# Autodesk Inventor assembly: hoops_sml_med_lrg
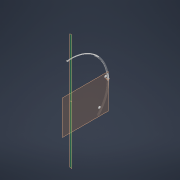
[picture p0: Inventor's stored thumbnail of the model, 180x180]
Saved by Autodesk Inventor 2021 (Build 250183000, 183)
## iProperties
Created: 2021-05-05
Part Number: hoops_sml_med_lrg
Document SubType Name: Assembly
## Documents named in this file (11)
- C:\Users\Watchdog\OneDrive - Flinders\Advn Mech Design Shared\6_Development\2_Design\inventor\Brandon_Hoop_specs\hoops_sml_med_lrg.iam
- C:\Users\Watchdog\OneDrive - Flinders\Advn Mech Design Shared\6_Development\2_Design\inventor\Brandon_Hoop_specs\large_hoop.ipt
- C:\Users\Watchdog\OneDrive - Flinders\Advn Mech Design Shared\6_Development\2_Design\inventor\Brandon_Hoop_specs\medium_hoop.ipt
- C:\Users\Watchdog\OneDrive - Flinders\Advn Mech Design Shared\6_Development\2_Design\inventor\rack_pinion\pinion.ipt
- C:\Users\Watchdog\OneDrive - Flinders\Advn Mech Design Shared\6_Development\2_Design\inventor\Brandon_Hoop_specs\small_hoop.ipt
- C:\Users\Watchdog\OneDrive - Flinders\Advn Mech Design Shared\6_Development\2_Design\inventor\rack_pinion\tooth.ipt
- C:\Users\Watchdog\OneDrive - Flinders\Advn Mech Design Shared\6_Development\2_Design\inventor\rack_pinion\pulley_guide.ipt
- C:\Users\Watchdog\OneDrive - Flinders\Advn Mech Design Shared\6_Development\2_Design\inventor\rack_pinion\large_bearings.ipt
- C:\Users\Watchdog\OneDrive - Flinders\Advn Mech Design Shared\6_Development\2_Design\inventor\rack_pinion\medium_bearings.ipt
- C:\Users\Watchdog\OneDrive - Flinders\Advn Mech Design Shared\6_Development\2_Design\inventor\rack_pinion\medium_pulley.ipt
- C:\Users\Watchdog\OneDrive - Flinders\Advn Mech Design Shared\6_Development\2_Design\inventor\params.xlsx
## Components (69 placed, 9 different names)
1. large_hoop:1 — Mate:1, Flush:1, Flush:12, Angle:1
2. medium_hoop:1 — Mate:2, Flush:2, Mate:4, Flush:8, Flush:9, Mate:6, Mate:7, Mate:12
3. pinion:1 — Flush:6
4. small_hoop:1 — Mate:3, Flush:7, Mate:8, Mate:9
5. large_bearings:1 — Mate:6, Flush:12
6. medium_bearings:1 — Flush:13, Mate:7
7. pinion:2
8. pulley_guide:1 — Mate:8, Mate:9, Mate:10
9. medium_pulley:1 — Mate:11, Mate:12
10. tooth:1 — Mate:4, Flush:8, Flush:9
11. tooth:2
12. tooth:3
13. tooth:4
14. tooth:5
15. tooth:6
16. tooth:7
17. tooth:8
18. tooth:9
19. tooth:10
20. tooth:11
21. tooth:12
22. tooth:13
23. tooth:14
24. tooth:15
25. tooth:16
26. tooth:17
27. tooth:18
28. tooth:19
29. tooth:20
30. tooth:21
31. tooth:22
32. tooth:23
33. tooth:24
34. tooth:25
35. tooth:26
36. tooth:27
37. tooth:28
38. tooth:29
39. tooth:30
40. tooth:31
41. tooth:32
42. tooth:33
43. tooth:34
44. tooth:35
45. tooth:36
46. tooth:37
47. tooth:38
48. tooth:39
49. tooth:40
50. tooth:41
51. tooth:42
52. tooth:43
53. tooth:44
54. tooth:45
55. tooth:46
56. tooth:47
57. tooth:48
58. tooth:49
59. tooth:50
60. tooth:51
61. tooth:52
62. tooth:53
63. tooth:54
64. tooth:55
65. tooth:56
66. tooth:57
67. tooth:58
68. tooth:59
69. tooth:60
## Component patterns: (60 elements, first: tooth:1)
## Relationships (21: Mate 11, Flush 9, Angle 1)
- Mate:1: large_hoop:1
- Mate:2: medium_hoop:1
- Flush:1: large_hoop:1
- Flush:2: medium_hoop:1
- Flush:6: pinion:1
- Mate:3: small_hoop:1
- Flush:7: small_hoop:1
- Mate:4: medium_hoop:1 ↔ tooth:1
- Flush:8: medium_hoop:1 ↔ tooth:1
- Flush:9: medium_hoop:1 ↔ tooth:1
- Mate:6: medium_hoop:1 ↔ large_bearings:1
- Flush:12: large_hoop:1 ↔ large_bearings:1
- Flush:13: medium_bearings:1
- Mate:7: medium_hoop:1 ↔ medium_bearings:1
- Mate:8 (-10 mm): small_hoop:1 ↔ pulley_guide:1
- Mate:9: small_hoop:1 ↔ pulley_guide:1
- Mate:10: pulley_guide:1
- Mate:11: medium_pulley:1
- Mate:12: medium_hoop:1 ↔ medium_pulley:1
- Flush:14
- Angle:1 (180 deg): large_hoop:1
## Named parameters: testLength = 1700 mm, testWidth = 1500 mm, testHeight = 1000 mm, rack_tooth_thickness = 5 mm, rack_tooth_face_widh = 10 mm, rack_tooth_addendum = 5 mm, rack_tooth_dedendum = 5 mm, hoop_radius_large = 3300 mm, hoop_width_large = 80 mm, hoop_thickness_large = 10 mm, hoop_width_medium = 60 mm, hoop_thickness_medium = 10 mm, hoop_width_small = 40 mm, hoop_thickness_small = 10 mm, hoop_height_large = 450 mm, hoop_height_medium = 450 mm, hoop_height_small = 600 mm, hoop_length_large = 200 mm, hoop_length_medium = 700 mm, hoop_length_small = 700 mm, cover_width_main = 1600 mm, cover_height_main = 900 mm, cover_length_main = 2200 mm, cover_shell_thickness = 10 mm, cover_base_thickness = 10 mm, cover_mountHole_diameter = 10 mm, cover_mountHole_xSpacing = 900 mm, cover_mountHole_ySpacing = 550 mm, cover_side_thickness = 20 mm, cover_side_openSize = 1400 mm, hoop_bearing_length = 5 deg, hoop_cable_diam = 5 mm, hoop_cable_pulley_diam = 22 mm, secure_arm_length = 400 mm, secure_arm_radii = 9 mm, secure_arm_hold_length = 35 mm, secure_arm_hold_thickness = 10 mm, secure_arm_thickness = 20 mm, secure_arm_angle = 20 deg, support_frame_squareBarThickness = 5 mm, support_frame_squareBarDimension = 50 mm, support_frame_squareBarFillet = 2 mm, support_baseClamp_platformThickness = 15 mm, support_baseClamp_sleeve_hole2Height = 100 mm, support_baseClamp_platformWidthBuffer = 0 mm, support_baseClamp_sleeveThickness = 20 mm, support_baseClamp_platformLengthBuffer = 35 mm, support_baseClamp_sleeve_hole1Height = 50 mm, support_frame_length = 500 mm, support_frame_endHoleBuffer = 25 mm, support_frame_clampHoleSpacing = 100 mm, support_frame_clampHoleDiameter = 10 mm, support_baseClamp_thickness = 8 mm, support_baseClamp_sleeveSweepTerminationAngle = 55 deg, support_baseClamp_sleeveHoleDiameter = 12 mm, support_baseClamp_lengthBuffer = 40 mm, hoop_offset_x = 600 mm, hoop_angle_z = 45 deg, hoop_tabs_hole = 12 mm, hoop_tabs_width = 50 mm, hoop_tabs_thickness = 6 mm, wheelchair_deployed_length = 1067 mm, wheelchair_deployed_height = 914 mm, wheelchair_wheel_radius = 240 mm, wheelchair_deployed_width = 635 mm, wheelchair_folded_width = 280 mm, sm_varx_member_tolerance = 0.5 mm, sm_varx_x = 50 mm, sm_varx_squareBarThickness = 2.5 mm, sm_varx_z = 160 mm, sm_varx_pinPlate_aspectRatio = 2, sm_varx_x_arms = 50 mm, sm_varx_pinPlate_holeDiameter = 5 mm, sm_varx_pinPlate_thickness = 5 mm, sm_varx_y = 250 mm, sm_varx_squareBarDimension = 30 mm
